# Autodesk Inventor assembly: 圆筒储弹仓装配1
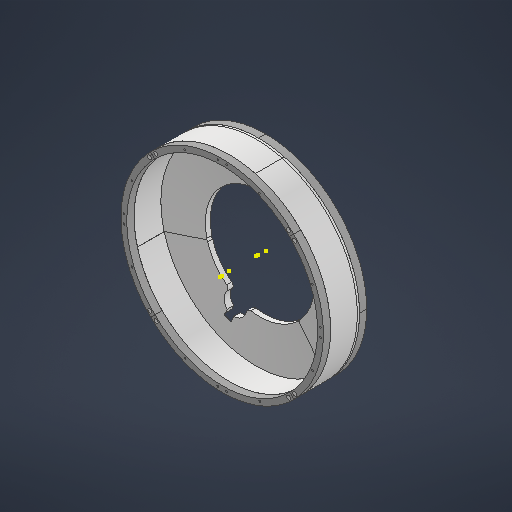
[picture p0: Inventor's stored thumbnail of the model, 512x512]
Saved by Autodesk Inventor 2025 (Build 290162000, 162)
## iProperties
Created: 2025-02-22
Part Number: 圆筒储弹仓装配1
Document SubType Name: Assembly
Designer: XH
Author: XH
## Documents named in this file (8)
- C:\1A_Engineering_files\GCG全向轮步兵\云台\圆筒储弹仓装配1.iam
- C:\1A_Engineering_files\GCG全向轮步兵\云台\零件149.ipt
- C:\1A_Engineering_files\GCG全向轮步兵\云台\零件1491.ipt
- C:\1A_Engineering_files\GCG全向轮步兵\云台\组合.ipt
- C:\1A_Engineering_files\GCG全向轮步兵\云台\零件149右.ipt
- C:\1A_Engineering_files\GCG全向轮步兵\云台\149后漏斗.ipt
- C:\1A_Engineering_files\GCG全向轮步兵\云台\149右漏斗.ipt
- C:\1A_Engineering_files\GCG全向轮步兵\云台\149左漏斗.ipt
## Components (14 placed, 7 different names)
1. 零件149:4 — 表面齐平:3, 配合:43, 配合:44, 配合:45, 配合:57, 配合:58, 配合:59, 配合:65
2. 零件1491:1 — 配合:48, 配合:49, 配合:50, 配合:70, 配合:71, 配合:74
3. 组合:1 — 表面齐平:1, 配合:36, 配合:37, 配合:41, 表面齐平:3, 配合:43, 配合:44
4. 组合:2 — 表面齐平:1, 配合:36, 配合:37, 配合:38, 配合:39, 表面齐平:2, 配合:46, 配合:47
5. 零件149右:1 — 配合:45, 配合:46, 配合:47, 配合:49, 配合:50, 配合:54, 配合:55, 配合:62, 配合:66, 配合:68
6. 组合:3 — 配合:38, 配合:39, 表面齐平:2, 配合:40, 配合:48
7. 组合:4 — 配合:40, 配合:41
8. 149右漏斗:1 — 配合:54, 配合:55, 配合:61, 配合:67
9. 149左漏斗:1 — 配合:57, 配合:58, 配合:59, 配合:60, 配合:63, 配合:64, 配合:73
10. 组合:5 — 配合:60, 配合:61, 配合:62
11. 组合:6 — 配合:63, 配合:64, 配合:65, 表面齐平:4
12. 组合:7 — 配合:66, 配合:67, 配合:68
13. 组合:8 — 配合:70, 配合:71, 配合:72, 表面齐平:4
14. 149后漏斗:1 — 配合:72, 配合:73, 配合:74
## Relationships (37: Mate 33, Flush 4)
- 表面齐平:1 [Flush]: 组合:1 ↔ 组合:2
- 配合:36 [Mate]: 组合:1 ↔ 组合:2
- 配合:37 [Mate]: 组合:1 ↔ 组合:2
- 配合:38 [Mate]: 组合:2 ↔ 组合:3
- 配合:39 [Mate]: 组合:2 ↔ 组合:3
- 表面齐平:2 [Flush]: 组合:2 ↔ 组合:3
- 配合:40 [Mate]: 组合:3 ↔ 组合:4
- 配合:41 [Mate]: 组合:1 ↔ 组合:4
- 表面齐平:3 [Flush]: 零件149:4 ↔ 组合:1
- 配合:43 [Mate]: 零件149:4 ↔ 组合:1
- 配合:44 [Mate]: 零件149:4 ↔ 组合:1
- 配合:45 [Mate]: 零件149:4 ↔ 零件149右:1
- 配合:46 [Mate]: 组合:2 ↔ 零件149右:1
- 配合:47 [Mate]: 组合:2 ↔ 零件149右:1
- 配合:48 [Mate]: 零件1491:1 ↔ 组合:3
- 配合:49 [Mate]: 零件1491:1 ↔ 零件149右:1
- 配合:50 [Mate]: 零件1491:1 ↔ 零件149右:1
- 配合:54 [Mate]: 零件149右:1 ↔ 149右漏斗:1
- 配合:55 [Mate]: 零件149右:1 ↔ 149右漏斗:1
- 配合:57 [Mate]: 零件149:4 ↔ 149左漏斗:1
- 配合:58 [Mate]: 零件149:4 ↔ 149左漏斗:1
- 配合:59 [Mate]: 零件149:4 ↔ 149左漏斗:1
- 配合:60 [Mate]: 149左漏斗:1 ↔ 组合:5
- 配合:61 [Mate]: 149右漏斗:1 ↔ 组合:5
- 配合:62 [Mate]: 零件149右:1 ↔ 组合:5
- 配合:63 [Mate]: 149左漏斗:1 ↔ 组合:6
- 配合:64 [Mate]: 149左漏斗:1 ↔ 组合:6
- 配合:65 [Mate]: 零件149:4 ↔ 组合:6
- 配合:66 [Mate]: 零件149右:1 ↔ 组合:7
- 配合:67 [Mate]: 149右漏斗:1 ↔ 组合:7
- 配合:68 [Mate]: 零件149右:1 ↔ 组合:7
- 配合:70 [Mate]: 零件1491:1 ↔ 组合:8
- 配合:71 [Mate]: 零件1491:1 ↔ 组合:8
- 配合:72 [Mate]: 组合:8 ↔ 149后漏斗:1
- 表面齐平:4 [Flush]: 组合:6 ↔ 组合:8
- 配合:73 [Mate]: 149左漏斗:1 ↔ 149后漏斗:1
- 配合:74 [Mate]: 零件1491:1 ↔ 149后漏斗:1
